# Autodesk Inventor assembly: PistonFeederHeadMini
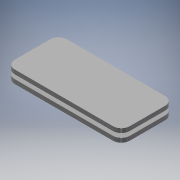
[picture p0: Inventor's stored thumbnail of the model, 180x180]
Saved by Autodesk Inventor 2016 (Build 200138000, 138)
## iProperties
Created: 2015-08-02
Part Number: PistonFeederHeadMini
Document SubType Name: Assembly
Designer: myhome
Author: myhome
## Documents named in this file (3)
- C:\Users\myhome\Documents\Inventor\Printer\PistonHead\PistonFeederHeadMini.iam
- C:\Users\myhome\Documents\Inventor\Printer\PistonHead\PistonFeederHeadMini.ipt
- C:\Users\myhome\Documents\Inventor\Printer\PistonHead\PistonFeederHeadInnerMini.ipt
## Components (3 placed, 2 different names)
1. PistonFeederHeadMini:1 — Rigid:1
2. PistonFeederHeadInnerMini:1 — Rigid:1, Rigid:2
3. PistonFeederHeadMini:2 — Rigid:2
## Relationships (2: WeldJoint 2)
- Rigid:1 [WeldJoint]: PistonFeederHeadMini:1 ↔ PistonFeederHeadInnerMini:1
- Rigid:2 [WeldJoint]: PistonFeederHeadInnerMini:1 ↔ PistonFeederHeadMini:2
